# Autodesk Inventor assembly: ConjuntoBracket2020
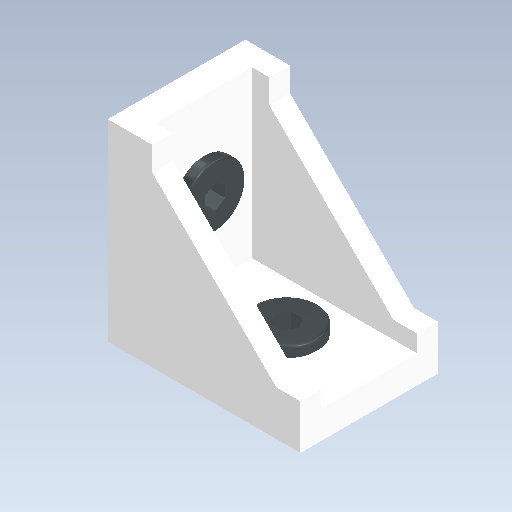
[picture p0: Inventor's stored thumbnail of the model, 512x512]
Saved by Autodesk Inventor 2020.2 (Build 242310000, 310)
## iProperties
Created: 2020-12-31
Part Number: ConjuntoBracket2020
Document SubType Name: Assembly
Designer: JK
Author: JK
## Documents named in this file (4)
- C:\Users\JK\Documents\Inventor\BioMixer\Chasis\ConjuntoUnion90GradosPerfil2020.iam
- C:\Users\JK\Documents\Inventor\BioMixer\Chasis\AnguloUnion90gradosPerfil2020.ipt
- C:\Users\JK\Documents\Inventor\BioMixer\Chasis\PernoM5x8Plano.ipt
- C:\Users\JK\Documents\Inventor\BioMixer\Chasis\TuercaTM5Perfil2020.ipt
## Components (5 placed, 3 different names)
1. AnguloUnion90gradosPerfil2020:1 — Mate:1, Mate:2, Mate:3, Mate:4, Angle:1, Mate:7, Mate:8, Angle:2, Angle:3
2. PernoM5x8Plano:1 — Mate:1, Mate:4, Mate:5
3. PernoM5x8Plano:2 — Mate:2, Mate:3, Mate:6
4. TuercaTM5Perfil2020:1 — Mate:6, Mate:7, Angle:3
5. TuercaTM5Perfil2020:2 — Mate:5, Angle:1, Mate:8, Angle:2
## Relationships (11: Mate 8, Angle 3)
- Mate:1: AnguloUnion90gradosPerfil2020:1 ↔ PernoM5x8Plano:1
- Mate:2: AnguloUnion90gradosPerfil2020:1 ↔ PernoM5x8Plano:2
- Mate:3: AnguloUnion90gradosPerfil2020:1 ↔ PernoM5x8Plano:2
- Mate:4: AnguloUnion90gradosPerfil2020:1 ↔ PernoM5x8Plano:1
- Mate:5: PernoM5x8Plano:1 ↔ TuercaTM5Perfil2020:2
- Mate:6: PernoM5x8Plano:2 ↔ TuercaTM5Perfil2020:1
- Angle:1 (0 deg): AnguloUnion90gradosPerfil2020:1 ↔ TuercaTM5Perfil2020:2
- Mate:7 (0.5 mm): AnguloUnion90gradosPerfil2020:1 ↔ TuercaTM5Perfil2020:1
- Mate:8 (0.5 mm): AnguloUnion90gradosPerfil2020:1 ↔ TuercaTM5Perfil2020:2
- Angle:2 (0 deg): AnguloUnion90gradosPerfil2020:1 ↔ TuercaTM5Perfil2020:2
- Angle:3 (0 deg): AnguloUnion90gradosPerfil2020:1 ↔ TuercaTM5Perfil2020:1
